# Autodesk Inventor assembly: Assemblage final
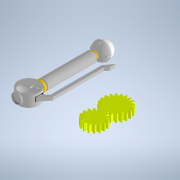
[picture p0: Inventor's stored thumbnail of the model, 180x180]
Saved by Autodesk Inventor 2021 (Build 250183000, 183)
## iProperties
Created: 2020-09-18
Part Number: Assemblage final
Document SubType Name: Assembly
Designer: Utilisateur
Author: Utilisateur
## Documents named in this file (13)
- F:\Projets Inventor\The long memory\Assemblage final - Copie.iam
- F:\Projets Inventor\The long memory\Anneau inf.ipt
- F:\Projets Inventor\The long memory\Anneau interm.ipt
- F:\Projets Inventor\The long memory\Manche interm.ipt
- F:\Projets Inventor\The long memory\Anneau sup.ipt
- F:\Projets Inventor\The long memory\Cadran base.ipt
- F:\Projets Inventor\The long memory\Cadran arriere cache.ipt
- F:\Projets Inventor\The long memory\Candran face cache.ipt
- F:\Projets Inventor\The long memory\Rouages.iam
- F:\Projets Inventor\The long memory\Cadre encoche manette.ipt
- F:\Projets Inventor\The long memory\Mannette.ipt
- F:\Projets Inventor\The long memory\Globe Pommeau.ipt
- F:\Projets Inventor\The long memory\Pommeau base.ipt
## Components (12 placed, 12 different names)
1. Anneau inf:1
2. Anneau interm:1 — Placage:3
3. Manche interm:1 — Placage:1, Placage:3
4. Anneau sup:1 — Placage:1
5. Cadran base:1 — Placage:2, Tangente:1
6. Cadran arriere cache:1
7. Candran face cache:1 — Placage:2
8. Rouages:1 [sub-assembly]
9. Cadre encoche manette:1
10. Mannette:1 — Tangente:1
11. Globe Pommeau:1
12. Pommeau base:1
## Relationships (4: Mate 3, Tangent 1)
- Placage:1 [Mate]: Manche interm:1 ↔ Anneau sup:1
- Placage:2 [Mate]: Cadran base:1 ↔ Candran face cache:1
- Tangente:1: Cadran base:1 ↔ Mannette:1
- Placage:3 [Mate]: Anneau interm:1 ↔ Manche interm:1
